# Autodesk Inventor assembly: Assembly
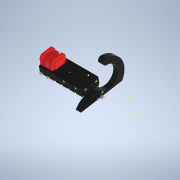
[picture p0: Inventor's stored thumbnail of the model, 180x180]
Saved by Autodesk Inventor 2022 (Build 260153000, 153)
## iProperties
Created: 2022-02-10
Part Number: Assembly
Document SubType Name: Assembly
Designer: br4ch
Author: br4ch
## Documents named in this file (19)
- C:\Users\br4ch\M-and-Ms\HW3\Inventor\Assembly.iam
- C:\Users\br4ch\M-and-Ms\HW3\Inventor\Pipka.ipt
- C:\Users\br4ch\M-and-Ms\HW3\Inventor\Plate.ipt
- C:\Users\br4ch\M-and-Ms\HW3\Inventor\Shaft box.ipt
- C:\Users\br4ch\M-and-Ms\HW3\Inventor\Shaft cap.ipt
- C:\Users\br4ch\M-and-Ms\HW3\Inventor\Shaft.ipt
- C:\Users\br4ch\M-and-Ms\HW3\Inventor\Spacer with a hole.ipt
- C:\Users\br4ch\M-and-Ms\HW3\Inventor\Spacer.ipt
- C:\Users\br4ch\M-and-Ms\HW3\Inventor\Current collector.ipt
- C:\Users\br4ch\M-and-Ms\HW3\Inventor\Disk lapka.ipt
- C:\Users\br4ch\M-and-Ms\HW3\Inventor\Disk.ipt
- C:\Users\br4ch\M-and-Ms\HW3\Inventor\lapka_80_double v3.ipt
- C:\Users\br4ch\M-and-Ms\HW3\Inventor\MX-28T_R v1.ipt
- C:\Users\br4ch\M-and-Ms\HW3\Inventor\bearing.ipt
- C:\Users\br4ch\M-and-Ms\HW3\Inventor\Plate_MIR.ipt
- C:\Users\br4ch\Documents\Inventor\Content Center Files\R2022\en-US\ANSI B18.6.5M(13)\ANSI B18.6.5M - M3x0,5 x 10(32).ipt
- C:\Users\br4ch\Documents\Inventor\Content Center Files\R2022\en-US\ANSI B18.6.5M(09)\ANSI B18.6.5M - M3x0,5 x 10(30).ipt
- C:\Users\br4ch\Documents\Inventor\Content Center Files\R2022\en-US\ANSI B18.6.5M(13)\ANSI B18.6.5M - M3x0,5 x 16(32).ipt
- C:\Users\br4ch\Documents\Inventor\Content Center Files\R2022\en-US\ANSI B18.6.5M(13)\ANSI B18.6.5M - M3x0,5 x 8(32).ipt
## Components (34 placed, 21 different names)
1. АНЦП.014.00.00.001 — Cylindrical:8, Mate:7, Mate:13
2. АНЦП.014.00.00.002 — Cylindrical:1, Angle:1, Cylindrical:2, Cylindrical:3, Mate:3, Cylindrical:4, Cylindrical:5, Cylindrical:6, Cylindrical:7, Mate:4, Cylindrical:8, Cylindrical:9, Cylindrical:12, Cylindrical:21
3. АНЦП.014.00.00.003 — Cylindrical:10, Mate:8, Angle:2, Mate:9, Symmetry:1, Mate:10, Mate:11, Symmetry:2, Cylindrical:13, Cylindrical:14, Mate:14, Cylindrical:15, Cylindrical:16, Mate:15
4. АНЦП.014.00.00.004 — Cylindrical:6, Mate:5, Angle:2, Mate:9, Symmetry:1, Symmetry:2, Mate:29, Mate:30, Mate:31, Mate:32
5. АНЦП.014.00.00.005 — Cylindrical:13, Cylindrical:14, Mate:14, Cylindrical:17, Angle:4, Mate:16, Angle:5, Cylindrical:18, Mate:17
6. АНЦП.014.00.00.005-01 — Cylindrical:15, Cylindrical:16, Mate:15, Cylindrical:19, Cylindrical:20, Angle:6, Angle:7, Mate:18, Mate:19
7. АНЦП.014.00.00.006 — Cylindrical:9, Mate:6, Mate:7
8. АНЦП.014.00.00.007 — Mate:12, Cylindrical:12, Mate:13
9. АНЦП.014.00.00.008 — Cylindrical:1, Angle:1, Cylindrical:2, Flush:1, Angle:3, Cylindrical:22, Mate:20
10. АНЦП.014.00.00.009 — Mate:3, Cylindrical:4, Cylindrical:5, Cylindrical:11
11. АНЦП.014.00.00.010 — Cylindrical:17, Angle:4, Mate:16
12. АНЦП.014.00.00.010-01 — Angle:5, Cylindrical:18, Mate:17
13. АНЦП.014.00.00.010-02 — Cylindrical:19, Angle:6, Mate:18
14. АНЦП.014.00.00.010-03 — Cylindrical:20, Angle:7, Mate:19
15. АНЦП.014.00.00.011 — Cylindrical:21, Cylindrical:22, Mate:20, Mate:33, Mate:34, Mate:35
16. MX-28T_R v1:1 — Cylindrical:11, Mate:10, Mate:11
17. Rolling bearing GB/T 7218-1995 Type FSN 70000-Z F 639-Z:1 — Cylindrical:3, Mate:5
18. Rolling bearing GB/T 7218-1995 Type FSN 70000-Z F 639-Z:2 — Cylindrical:7, Mate:4, Mate:6, Cylindrical:10, Mate:8
19. Cross Recessed Flat Countersunk Head Tapping Screw - Type T - Type IA - Metric M3x0,5 x 10:2
20. Cross Recessed Flat Countersunk Head Tapping Screw - Type D - Type IA - Metric M3x0,5 x 10:1
21. Cross Recessed Flat Countersunk Head Tapping Screw - Type D - Type IA - Metric M3x0,5 x 10:2
22. Cross Recessed Flat Countersunk Head Tapping Screw - Type D - Type IA - Metric M3x0,5 x 10:3
23. Cross Recessed Flat Countersunk Head Tapping Screw - Type D - Type IA - Metric M3x0,5 x 10:4
24. Cross Recessed Flat Countersunk Head Tapping Screw - Type D - Type IA - Metric M3x0,5 x 10:5
25. Cross Recessed Flat Countersunk Head Tapping Screw - Type D - Type IA - Metric M3x0,5 x 10:6
26. Cross Recessed Flat Countersunk Head Tapping Screw - Type D - Type IA - Metric M3x0,5 x 10:7
27. Cross Recessed Flat Countersunk Head Tapping Screw - Type D - Type IA - Metric M3x0,5 x 10:8
28. Cross Recessed Flat Countersunk Head Tapping Screw - Type T - Type IA - Metric M3x0,5 x 8:1 — Mate:29
29. Cross Recessed Flat Countersunk Head Tapping Screw - Type T - Type IA - Metric M3x0,5 x 8:4 — Mate:30
30. Cross Recessed Flat Countersunk Head Tapping Screw - Type T - Type IA - Metric M3x0,5 x 8:2 — Mate:31
31. Cross Recessed Flat Countersunk Head Tapping Screw - Type T - Type IA - Metric M3x0,5 x 8:3 — Mate:32
32. Cross Recessed Flat Countersunk Head Tapping Screw - Type T - Type IA - Metric M3x0,5 x 16:3 — Mate:33
33. Cross Recessed Flat Countersunk Head Tapping Screw - Type T - Type IA - Metric M3x0,5 x 16:1 — Mate:34
34. Cross Recessed Flat Countersunk Head Tapping Screw - Type T - Type IA - Metric M3x0,5 x 16:2 — Mate:35
## Relationships (65: Mate 33, CylindricalJoint 22, Angle 7, Symmetry 2, Flush 1)
- Cylindrical:1: АНЦП.014.00.00.002 ↔ АНЦП.014.00.00.008
- Angle:1 (0 deg): АНЦП.014.00.00.002 ↔ АНЦП.014.00.00.008
- Cylindrical:2: АНЦП.014.00.00.002 ↔ АНЦП.014.00.00.008
- Flush:1: АНЦП.014.00.00.008
- Cylindrical:3: АНЦП.014.00.00.002 ↔ Rolling bearing GB/T 7218-1995 Type FSN 70000-Z F 639-Z:1
- Mate:3: АНЦП.014.00.00.002 ↔ АНЦП.014.00.00.009
- Cylindrical:4: АНЦП.014.00.00.002 ↔ АНЦП.014.00.00.009
- Cylindrical:5: АНЦП.014.00.00.002 ↔ АНЦП.014.00.00.009
- Cylindrical:6: АНЦП.014.00.00.002 ↔ АНЦП.014.00.00.004
- Cylindrical:7: АНЦП.014.00.00.002 ↔ Rolling bearing GB/T 7218-1995 Type FSN 70000-Z F 639-Z:2
- Mate:4: АНЦП.014.00.00.002 ↔ Rolling bearing GB/T 7218-1995 Type FSN 70000-Z F 639-Z:2
- Mate:5: АНЦП.014.00.00.004 ↔ Rolling bearing GB/T 7218-1995 Type FSN 70000-Z F 639-Z:1
- Cylindrical:8: АНЦП.014.00.00.001 ↔ АНЦП.014.00.00.002
- Cylindrical:9: АНЦП.014.00.00.002 ↔ АНЦП.014.00.00.006
- Mate:6: АНЦП.014.00.00.006 ↔ Rolling bearing GB/T 7218-1995 Type FSN 70000-Z F 639-Z:2
- Mate:7: АНЦП.014.00.00.001 ↔ АНЦП.014.00.00.006
- Cylindrical:10: АНЦП.014.00.00.003 ↔ Rolling bearing GB/T 7218-1995 Type FSN 70000-Z F 639-Z:2
- Mate:8: АНЦП.014.00.00.003 ↔ Rolling bearing GB/T 7218-1995 Type FSN 70000-Z F 639-Z:2
- Angle:2 (0 deg): АНЦП.014.00.00.003 ↔ АНЦП.014.00.00.004
- Mate:9: АНЦП.014.00.00.003 ↔ АНЦП.014.00.00.004
- Symmetry:1: АНЦП.014.00.00.003 ↔ АНЦП.014.00.00.004
- Angle:3 (0 deg): АНЦП.014.00.00.008
- Cylindrical:11: АНЦП.014.00.00.009 ↔ MX-28T_R v1:1
- Mate:10: АНЦП.014.00.00.003 ↔ MX-28T_R v1:1
- Mate:11: АНЦП.014.00.00.003 ↔ MX-28T_R v1:1
- Symmetry:2: АНЦП.014.00.00.003 ↔ АНЦП.014.00.00.004
- Mate:12: АНЦП.014.00.00.007
- Cylindrical:12: АНЦП.014.00.00.002 ↔ АНЦП.014.00.00.007
- Mate:13: АНЦП.014.00.00.001 ↔ АНЦП.014.00.00.007
- Cylindrical:13: АНЦП.014.00.00.003 ↔ АНЦП.014.00.00.005
- Cylindrical:14: АНЦП.014.00.00.003 ↔ АНЦП.014.00.00.005
- Mate:14: АНЦП.014.00.00.003 ↔ АНЦП.014.00.00.005
- Cylindrical:15: АНЦП.014.00.00.003 ↔ АНЦП.014.00.00.005-01
- Cylindrical:16: АНЦП.014.00.00.003 ↔ АНЦП.014.00.00.005-01
- Mate:15: АНЦП.014.00.00.003 ↔ АНЦП.014.00.00.005-01
- Cylindrical:17: АНЦП.014.00.00.005 ↔ АНЦП.014.00.00.010
- Angle:4 (0 deg): АНЦП.014.00.00.005 ↔ АНЦП.014.00.00.010
- Mate:16: АНЦП.014.00.00.005 ↔ АНЦП.014.00.00.010
- Angle:5 (0 deg): АНЦП.014.00.00.005 ↔ АНЦП.014.00.00.010-01
- Cylindrical:18: АНЦП.014.00.00.005 ↔ АНЦП.014.00.00.010-01
- Mate:17: АНЦП.014.00.00.005 ↔ АНЦП.014.00.00.010-01
- Cylindrical:19: АНЦП.014.00.00.005-01 ↔ АНЦП.014.00.00.010-02
- Cylindrical:20: АНЦП.014.00.00.005-01 ↔ АНЦП.014.00.00.010-03
- Angle:6 (0 deg): АНЦП.014.00.00.005-01 ↔ АНЦП.014.00.00.010-02
- Angle:7 (0 deg): АНЦП.014.00.00.005-01 ↔ АНЦП.014.00.00.010-03
- Mate:18: АНЦП.014.00.00.005-01 ↔ АНЦП.014.00.00.010-02
- Mate:19: АНЦП.014.00.00.005-01 ↔ АНЦП.014.00.00.010-03
- Cylindrical:21: АНЦП.014.00.00.002 ↔ АНЦП.014.00.00.011
- Cylindrical:22: АНЦП.014.00.00.008 ↔ АНЦП.014.00.00.011
- Mate:20: АНЦП.014.00.00.008 ↔ АНЦП.014.00.00.011
- [Mate]: АНЦП.014.00.00.005-01 ↔ Cross Recessed Flat Countersunk Head Tapping Screw - Type D - Type IA - Metric M3x0,5 x 10:1
- [Mate]: АНЦП.014.00.00.005-01 ↔ Cross Recessed Flat Countersunk Head Tapping Screw - Type D - Type IA - Metric M3x0,5 x 10:2
- [Mate]: АНЦП.014.00.00.005-01 ↔ Cross Recessed Flat Countersunk Head Tapping Screw - Type D - Type IA - Metric M3x0,5 x 10:3
- [Mate]: АНЦП.014.00.00.005-01 ↔ Cross Recessed Flat Countersunk Head Tapping Screw - Type D - Type IA - Metric M3x0,5 x 10:4
- [Mate]: АНЦП.014.00.00.005 ↔ Cross Recessed Flat Countersunk Head Tapping Screw - Type D - Type IA - Metric M3x0,5 x 10:5
- [Mate]: АНЦП.014.00.00.005 ↔ Cross Recessed Flat Countersunk Head Tapping Screw - Type D - Type IA - Metric M3x0,5 x 10:6
- [Mate]: АНЦП.014.00.00.005 ↔ Cross Recessed Flat Countersunk Head Tapping Screw - Type D - Type IA - Metric M3x0,5 x 10:7
- [Mate]: АНЦП.014.00.00.005 ↔ Cross Recessed Flat Countersunk Head Tapping Screw - Type D - Type IA - Metric M3x0,5 x 10:8
- Mate:29: АНЦП.014.00.00.004 ↔ Cross Recessed Flat Countersunk Head Tapping Screw - Type T - Type IA - Metric M3x0,5 x 8:1
- Mate:30: АНЦП.014.00.00.004 ↔ Cross Recessed Flat Countersunk Head Tapping Screw - Type T - Type IA - Metric M3x0,5 x 8:4
- Mate:31: АНЦП.014.00.00.004 ↔ Cross Recessed Flat Countersunk Head Tapping Screw - Type T - Type IA - Metric M3x0,5 x 8:2
- Mate:32: АНЦП.014.00.00.004 ↔ Cross Recessed Flat Countersunk Head Tapping Screw - Type T - Type IA - Metric M3x0,5 x 8:3
- Mate:33: АНЦП.014.00.00.011 ↔ Cross Recessed Flat Countersunk Head Tapping Screw - Type T - Type IA - Metric M3x0,5 x 16:3
- Mate:34: АНЦП.014.00.00.011 ↔ Cross Recessed Flat Countersunk Head Tapping Screw - Type T - Type IA - Metric M3x0,5 x 16:1
- Mate:35: АНЦП.014.00.00.011 ↔ Cross Recessed Flat Countersunk Head Tapping Screw - Type T - Type IA - Metric M3x0,5 x 16:2
